# Autodesk Inventor assembly: 110033226_iam_02_造型房屋一
(part 2 of 2)
- 貼合:33 [Mate]: 110033226_ipt_06_磚塊樺木(1x1):1 ↔ 110033226_ipt_07_磚塊樺木(2x1):18
- 貼合:34 [Mate]: 110033226_ipt_07_磚塊樺木(2x1):23 ↔ 110033226_ipt_06_磚塊樺木(1x1):17
- 貼合:35 [Mate]: 110033226_ipt_07_磚塊樺木(2x1):23 ↔ 110033226_ipt_06_磚塊樺木(1x1):17
- 貼合:36 [Mate]: 110033226_ipt_07_磚塊樺木(2x1):23 ↔ 110033226_ipt_07_磚塊樺木(2x1):18
- 貼合:37 [Mate]: 110033226_ipt_06_磚塊樺木(1x1):22 ↔ 110033226_ipt_07_磚塊樺木(2x1):18
- 貼合:38 [Mate]: 110033226_ipt_06_磚塊樺木(1x1):22 ↔ 110033226_ipt_07_磚塊樺木(2x1):18
- 貼合:39 [Mate]: 110033226_ipt_07_磚塊樺木(2x1):25 ↔ 110033226_ipt_06_磚塊樺木(1x1):19
- 貼合:40 [Mate]: 110033226_ipt_07_磚塊樺木(2x1):25 ↔ 110033226_ipt_06_磚塊樺木(1x1):19
- 貼合:41 [Mate]: 110033226_ipt_06_磚塊樺木(1x1):24 ↔ 110033226_ipt_07_磚塊樺木(2x1):20
- 貼合:42 [Mate]: 110033226_ipt_06_磚塊樺木(1x1):24 ↔ 110033226_ipt_07_磚塊樺木(2x1):20
- 貼合:43 [Mate]: 110033226_ipt_06_磚塊樺木(1x1):2 ↔ 110033226_ipt_07_磚塊樺木(2x1):21
- 貼合:44 [Mate]: 110033226_ipt_07_磚塊樺木(2x1):2 ↔ 110033226_ipt_06_磚塊樺木(1x1):25
- 貼合:45 [Mate]: 110033226_ipt_06_磚塊樺木(1x1):2 ↔ 110033226_ipt_07_磚塊樺木(2x1):21
- 貼合:46 [Mate]: 110033226_ipt_07_磚塊樺木(2x1):2 ↔ 110033226_ipt_07_磚塊樺木(2x1):21
- 貼合:47 [Mate]: 110033226_ipt_07_磚塊樺木(2x1):2 ↔ 110033226_ipt_06_磚塊樺木(1x1):25
- 貼合:48 [Mate]: 110033226_ipt_06_磚塊樺木(1x1):10 ↔ 110033226_ipt_07_磚塊樺木(2x1):22
- 貼合:49 [Mate]: 110033226_ipt_07_磚塊樺木(2x1):10 ↔ 110033226_ipt_07_磚塊樺木(2x1):22
- 貼合:50 [Mate]: 110033226_ipt_06_磚塊樺木(1x1):10 ↔ 110033226_ipt_07_磚塊樺木(2x1):22
- 貼合:51 [Mate]: 110033226_ipt_06_磚塊樺木(1x1):25 ↔ 110033226_ipt_07_磚塊樺木(2x1):24
- 貼合:52 [Mate]: 110033226_ipt_06_磚塊樺木(1x1):25 ↔ 110033226_ipt_07_磚塊樺木(2x1):24
- 貼合:53 [Mate]: 110033226_ipt_07_磚塊樺木(2x1):21 ↔ 110033226_ipt_07_磚塊樺木(2x1):24
- 貼合:54 [Mate]: 110033226_ipt_07_磚塊樺木(2x1):10 ↔ 110033226_ipt_06_磚塊樺木(1x1):20
- 貼合:55 [Mate]: 110033226_ipt_07_磚塊樺木(2x1):10 ↔ 110033226_ipt_06_磚塊樺木(1x1):20
- 貼合:56 [Mate]: 110033226_ipt_07_磚塊樺木(2x1):21 ↔ 110033226_ipt_06_磚塊樺木(1x1):21
- 貼合:57 [Mate]: 110033226_ipt_07_磚塊樺木(2x1):21 ↔ 110033226_ipt_06_磚塊樺木(1x1):21
- 貼合:58 [Mate]: 110033226_ipt_06_磚塊樺木(1x1):22 ↔ 110033226_ipt_07_磚塊樺木(2x1):26
- 貼合:59 [Mate]: 110033226_ipt_06_磚塊樺木(1x1):22 ↔ 110033226_ipt_07_磚塊樺木(2x1):26
- 貼合:60 [Mate]: 110033226_ipt_07_磚塊樺木(2x1):23 ↔ 110033226_ipt_07_磚塊樺木(2x1):26
- 貼合:61 [Mate]: 110033226_ipt_07_磚塊樺木(2x1):23 ↔ 110033226_ipt_06_磚塊樺木(1x1):23
- 貼合:62 [Mate]: 110033226_ipt_07_磚塊樺木(2x1):23 ↔ 110033226_ipt_06_磚塊樺木(1x1):23
- 貼合:63 [Mate]: 110033226_ipt_06_磚塊樺木(1x1):20 ↔ 110033226_ipt_07_磚塊樺木(2x1):46
- 貼合:64 [Mate]: 110033226_ipt_06_磚塊樺木(1x1):20 ↔ 110033226_ipt_07_磚塊樺木(2x1):46
- 貼合:65 [Mate]: 110033226_ipt_07_磚塊樺木(2x1):22 ↔ 110033226_ipt_07_磚塊樺木(2x1):46
- 貼合:66 [Mate]: 110033226_ipt_07_磚塊樺木(2x1):22 ↔ 110033226_ipt_06_磚塊樺木(1x1):43
- 貼合:67 [Mate]: 110033226_ipt_07_磚塊樺木(2x1):22 ↔ 110033226_ipt_06_磚塊樺木(1x1):43
- 貼合:68 [Mate]: 110033226_ipt_06_磚塊樺木(1x1):24 ↔ 110033226_ipt_07_磚塊樺木(2x1):25
- 貼合:69 [Mate]: 110033226_ipt_06_磚塊樺木(1x1):22 ↔ 110033226_ipt_06_磚塊樺木(1x1):18
- 貼合:70 [Mate]: 110033226_ipt_06_磚塊樺木(1x1):17 ↔ 110033226_ipt_07_磚塊樺木(2x1):18
- 貼合:71 [Mate]: 110033226_ipt_06_磚塊樺木(1x1):23 ↔ 110033226_ipt_07_磚塊樺木(2x1):26
- 貼合:72 [Mate]: 110033226_ipt_06_磚塊樺木(1x1):43 ↔ 110033226_ipt_07_磚塊樺木(2x1):46
- 貼合:73 [Mate]: 110033226_ipt_07_磚塊樺木(2x1):46 ↔ 110033226_ipt_06_磚塊樺木(1x1):42
- 貼合:74 [Mate]: 110033226_ipt_07_磚塊樺木(2x1):46 ↔ 110033226_ipt_06_磚塊樺木(1x1):42
- 貼合:75 [Mate]: 110033226_ipt_07_磚塊樺木(2x1):46 ↔ 110033226_ipt_07_磚塊樺木(2x1):44
- 貼合:76 [Mate]: 110033226_ipt_07_磚塊樺木(2x1):46 ↔ 110033226_ipt_07_磚塊樺木(2x1):44
- 貼合:77 [Mate]: 110033226_ipt_06_磚塊樺木(1x1):43 ↔ 110033226_ipt_07_磚塊樺木(2x1):44
- 貼合:78 [Mate]: 110033226_ipt_07_磚塊樺木(2x1):44 ↔ 110033226_ipt_06_磚塊樺木(1x1):42
- 貼合:79 [Mate]: 110033226_ipt_06_磚塊樺木(1x1):42 ↔ 110033226_ipt_07_磚塊樺木(2x1):43
- 貼合:80 [Mate]: 110033226_ipt_07_磚塊樺木(2x1):44 ↔ 110033226_ipt_07_磚塊樺木(2x1):43
- 貼合:81 [Mate]: 110033226_ipt_06_磚塊樺木(1x1):42 ↔ 110033226_ipt_07_磚塊樺木(2x1):43
- 貼合:82 [Mate]: 110033226_ipt_07_磚塊樺木(2x1):44 ↔ 110033226_ipt_06_磚塊樺木(1x1):44
- 貼合:83 [Mate]: 110033226_ipt_07_磚塊樺木(2x1):44 ↔ 110033226_ipt_06_磚塊樺木(1x1):44
- 貼合:84 [Mate]: 110033226_ipt_07_磚塊樺木(2x1):43 ↔ 110033226_ipt_07_磚塊樺木(2x1):45
- 貼合:85 [Mate]: 110033226_ipt_07_磚塊樺木(2x1):43 ↔ 110033226_ipt_07_磚塊樺木(2x1):45
- 貼合:86 [Mate]: 110033226_ipt_06_磚塊樺木(1x1):44 ↔ 110033226_ipt_07_磚塊樺木(2x1):45
- 貼合:87 [Mate]: 110033226_ipt_06_磚塊樺木(1x1):62 ↔ 110033226_ipt_07_磚塊樺木(2x1):52
- 貼合:88 [Mate]: 110033226_ipt_07_磚塊樺木(2x1):63 ↔ 110033226_ipt_07_磚塊樺木(2x1):52
- 貼合:89 [Mate]: 110033226_ipt_06_磚塊樺木(1x1):62 ↔ 110033226_ipt_07_磚塊樺木(2x1):52
- 貼合:93 [Mate]: 110033226_ipt_08_平滑面(3x1):3 ↔ 110033226_ipt_07_磚塊樺木(2x1):19
- 貼合:94 [Mate]: 110033226_ipt_08_平滑面(3x1):3 ↔ 110033226_ipt_07_磚塊樺木(2x1):19
- 貼合:95 [Mate]: 110033226_ipt_08_平滑面(3x1):3 ↔ 110033226_ipt_06_磚塊樺木(1x1):18
- 貼合:96 [Mate]: 110033226_ipt_07_磚塊樺木(2x1):63 ↔ 110033226_ipt_06_磚塊樺木(1x1):45
- 貼合:97 [Mate]: 110033226_ipt_07_磚塊樺木(2x1):63 ↔ 110033226_ipt_06_磚塊樺木(1x1):45
- 貼合:98 [Mate]: 110033226_ipt_07_磚塊樺木(2x1):52 ↔ 110033226_ipt_06_磚塊樺木(1x1):45
- 貼合:99 [Mate]: 110033226_ipt_07_磚塊樺木(2x1):52 ↔ 110033226_ipt_07_磚塊樺木(2x1):51
- 貼合:100 [Mate]: 110033226_ipt_06_磚塊樺木(1x1):45 ↔ 110033226_ipt_07_磚塊樺木(2x1):51
- 貼合:101 [Mate]: 110033226_ipt_07_磚塊樺木(2x1):52 ↔ 110033226_ipt_07_磚塊樺木(2x1):51
- 貼合:102 [Mate]: 110033226_ipt_07_磚塊樺木(2x1):43 ↔ 110033226_ipt_06_磚塊樺木(1x1):51
- 貼合:103 [Mate]: 110033226_ipt_07_磚塊樺木(2x1):43 ↔ 110033226_ipt_06_磚塊樺木(1x1):51
- 貼合:104 [Mate]: 110033226_ipt_07_磚塊樺木(2x1):51 ↔ 110033226_ipt_06_磚塊樺木(1x1):51
- 貼合:105 [Mate]: 110033226_ipt_07_磚塊樺木(2x1):52 ↔ 110033226_ipt_06_磚塊樺木(1x1):47
- 貼合:106 [Mate]: 110033226_ipt_07_磚塊樺木(2x1):52 ↔ 110033226_ipt_06_磚塊樺木(1x1):47
- 貼合:107 [Mate]: 110033226_ipt_06_磚塊樺木(1x1):47 ↔ 110033226_ipt_07_磚塊樺木(2x1):51
- 貼合:111 [Mate]: 110033226_ipt_07_磚塊樺木(2x1):51 ↔ 110033226_ipt_07_磚塊樺木(2x1):47
- 貼合:112 [Mate]: 110033226_ipt_07_磚塊樺木(2x1):51 ↔ 110033226_ipt_07_磚塊樺木(2x1):47
- 貼合:113 [Mate]: 110033226_ipt_06_磚塊樺木(1x1):47 ↔ 110033226_ipt_07_磚塊樺木(2x1):47
- 貼合:114 [Mate]: 110033226_ipt_07_磚塊樺木(2x1):51 ↔ 110033226_ipt_06_磚塊樺木(1x1):46
- 貼合:115 [Mate]: 110033226_ipt_07_磚塊樺木(2x1):51 ↔ 110033226_ipt_06_磚塊樺木(1x1):46
- 貼合:116 [Mate]: 110033226_ipt_07_磚塊樺木(2x1):47 ↔ 110033226_ipt_06_磚塊樺木(1x1):46
- 貼合:117 [Mate]: 110033226_ipt_09_窗戶圓拱:1 ↔ 110033226_ipt_07_磚塊樺木(2x1):47
- 貼合:118 [Mate]: 110033226_ipt_09_窗戶圓拱:1 ↔ 110033226_ipt_06_磚塊樺木(1x1):65
- 貼合:119 [Mate]: 110033226_ipt_09_窗戶圓拱:1 ↔ 110033226_ipt_06_磚塊樺木(1x1):65
- 貼合:120 [Mate]: 110033226_ipt_06_磚塊樺木(1x1):51 ↔ 110033226_ipt_07_磚塊樺木(2x1):49
- 貼合:121 [Mate]: 110033226_ipt_06_磚塊樺木(1x1):51 ↔ 110033226_ipt_07_磚塊樺木(2x1):49
- 貼合:122 [Mate]: 110033226_ipt_07_磚塊樺木(2x1):49 ↔ 110033226_ipt_07_磚塊樺木(2x1):45
- 貼合:123 [Mate]: 110033226_ipt_06_磚塊樺木(1x1):48 ↔ 110033226_ipt_07_磚塊樺木(2x1):45
- 貼合:124 [Mate]: 110033226_ipt_06_磚塊樺木(1x1):48 ↔ 110033226_ipt_07_磚塊樺木(2x1):45
- 貼合:125 [Mate]: 110033226_ipt_07_磚塊樺木(2x1):49 ↔ 110033226_ipt_06_磚塊樺木(1x1):48
- 貼合:126 [Mate]: 110033226_ipt_06_磚塊樺木(1x1):48 ↔ 110033226_ipt_07_磚塊樺木(2x1):70
- 貼合:127 [Mate]: 110033226_ipt_07_磚塊樺木(2x1):49 ↔ 110033226_ipt_07_磚塊樺木(2x1):70
- 貼合:128 [Mate]: 110033226_ipt_06_磚塊樺木(1x1):48 ↔ 110033226_ipt_07_磚塊樺木(2x1):70
- 貼合:129 [Mate]: 110033226_ipt_07_磚塊樺木(2x1):49 ↔ 110033226_ipt_06_磚塊樺木(1x1):74
- 貼合:130 [Mate]: 110033226_ipt_06_磚塊樺木(1x1):74 ↔ 110033226_ipt_07_磚塊樺木(2x1):70
- 貼合:131 [Mate]: 110033226_ipt_07_磚塊樺木(2x1):49 ↔ 110033226_ipt_06_磚塊樺木(1x1):74
- 貼合:132 [Mate]: 110033226_ipt_06_磚塊樺木(1x1):46 ↔ 110033226_ipt_07_磚塊樺木(2x1):75
- 貼合:133 [Mate]: 110033226_ipt_06_磚塊樺木(1x1):46 ↔ 110033226_ipt_07_磚塊樺木(2x1):75
- 貼合:134 [Mate]: 110033226_ipt_07_磚塊樺木(2x1):47 ↔ 110033226_ipt_07_磚塊樺木(2x1):75
- 貼合:135 [Mate]: 110033226_ipt_06_磚塊樺木(1x1):74 ↔ 110033226_ipt_07_磚塊樺木(2x1):79
- 貼合:136 [Mate]: 110033226_ipt_06_磚塊樺木(1x1):74 ↔ 110033226_ipt_07_磚塊樺木(2x1):79
- 貼合:137 [Mate]: 110033226_ipt_07_磚塊樺木(2x1):79 ↔ 110033226_ipt_07_磚塊樺木(2x1):70
- 貼合:138 [Mate]: 110033226_ipt_06_磚塊樺木(1x1):76 ↔ 110033226_ipt_07_磚塊樺木(2x1):70
- 貼合:139 [Mate]: 110033226_ipt_06_磚塊樺木(1x1):76 ↔ 110033226_ipt_07_磚塊樺木(2x1):70
- 貼合:140 [Mate]: 110033226_ipt_07_磚塊樺木(2x1):79 ↔ 110033226_ipt_06_磚塊樺木(1x1):76
- 貼合:141 [Mate]: 110033226_ipt_07_磚塊樺木(2x1):75 ↔ 110033226_ipt_07_磚塊樺木(2x1):78
- 貼合:142 [Mate]: 110033226_ipt_07_磚塊樺木(2x1):75 ↔ 110033226_ipt_07_磚塊樺木(2x1):78
- 貼合:143 [Mate]: 110033226_ipt_07_磚塊樺木(2x1):75 ↔ 110033226_ipt_07_磚塊樺木(2x1):78
- 貼合:144 [Mate]: 110033226_ipt_07_磚塊樺木(2x1):78 ↔ 110033226_ipt_07_磚塊樺木(2x1):73
- 貼合:145 [Mate]: 110033226_ipt_07_磚塊樺木(2x1):78 ↔ 110033226_ipt_07_磚塊樺木(2x1):73
- 貼合:146 [Mate]: 110033226_ipt_07_磚塊樺木(2x1):78 ↔ 110033226_ipt_07_磚塊樺木(2x1):73
- 貼合:147 [Mate]: 110033226_ipt_07_磚塊樺木(2x1):73 ↔ 110033226_ipt_07_磚塊樺木(2x1):72
- 貼合:148 [Mate]: 110033226_ipt_07_磚塊樺木(2x1):73 ↔ 110033226_ipt_07_磚塊樺木(2x1):72
- 貼合:149 [Mate]: 110033226_ipt_07_磚塊樺木(2x1):73 ↔ 110033226_ipt_07_磚塊樺木(2x1):72
- 貼合:150 [Mate]: 110033226_ipt_07_磚塊樺木(2x1):72 ↔ 110033226_ipt_06_磚塊樺木(1x1):71
- 貼合:151 [Mate]: 110033226_ipt_07_磚塊樺木(2x1):72 ↔ 110033226_ipt_06_磚塊樺木(1x1):71
- 貼合:152 [Mate]: 110033226_ipt_09_窗戶圓拱:1 ↔ 110033226_ipt_07_磚塊樺木(2x1):74
- 貼合:153 [Mate]: 110033226_ipt_07_磚塊樺木(2x1):72 ↔ 110033226_ipt_07_磚塊樺木(2x1):74
- 貼合:154 [Mate]: 110033226_ipt_07_磚塊樺木(2x1):74 ↔ 110033226_ipt_06_磚塊樺木(1x1):71
- 貼合:155 [Mate]: 110033226_ipt_07_磚塊樺木(2x1):74 ↔ 110033226_ipt_08_平滑面(3x1):2
- 貼合:156 [Mate]: 110033226_ipt_06_磚塊樺木(1x1):71 ↔ 110033226_ipt_08_平滑面(3x1):2
- 貼合:157 [Mate]: 110033226_ipt_07_磚塊樺木(2x1):74 ↔ 110033226_ipt_08_平滑面(3x1):2
- 對稱:1 [Symmetry]: 110033226_ipt_06_磚塊樺木(1x1):76 ↔ 110033226_ipt_07_磚塊樺木(2x1):67
- 貼合:158 [Mate]: 110033226_ipt_07_磚塊樺木(2x1):79 ↔ 110033226_ipt_07_磚塊樺木(2x1):67
- 貼合:159 [Mate]: 110033226_ipt_06_磚塊樺木(1x1):76 ↔ 110033226_ipt_07_磚塊樺木(2x1):67
- 貼合:160 [Mate]: 110033226_ipt_07_磚塊樺木(2x1):79 ↔ 110033226_ipt_06_磚塊樺木(1x1):69
- 貼合:161 [Mate]: 110033226_ipt_07_磚塊樺木(2x1):79 ↔ 110033226_ipt_06_磚塊樺木(1x1):69
- 角度:1 [Angle] (0 deg): 110033226_ipt_07_磚塊樺木(2x1):67 ↔ 110033226_ipt_06_磚塊樺木(1x1):69
- 貼合:162 [Mate]: 110033226_ipt_07_磚塊樺木(2x1):71 ↔ 110033226_ipt_06_磚塊樺木(1x1):69
- 貼合:163 [Mate]: 110033226_ipt_07_磚塊樺木(2x1):67 ↔ 110033226_ipt_07_磚塊樺木(2x1):71
- 貼合:164 [Mate]: 110033226_ipt_07_磚塊樺木(2x1):71 ↔ 110033226_ipt_06_磚塊樺木(1x1):69
- 貼合:165 [Mate]: 110033226_ipt_07_磚塊樺木(2x1):67 ↔ 110033226_ipt_06_磚塊樺木(1x1):70
- 貼合:166 [Mate]: 110033226_ipt_07_磚塊樺木(2x1):67 ↔ 110033226_ipt_06_磚塊樺木(1x1):70
- 貼合:167 [Mate]: 110033226_ipt_06_磚塊樺木(1x1):70 ↔ 110033226_ipt_07_磚塊樺木(2x1):71
- 貼合:168 [Mate]: 110033226_ipt_06_磚塊樺木(1x1):70 ↔ 110033226_ipt_08_平滑面(3x1):5
- 貼合:169 [Mate]: 110033226_ipt_07_磚塊樺木(2x1):71 ↔ 110033226_ipt_08_平滑面(3x1):5
- 貼合:170 [Mate]: 110033226_ipt_06_磚塊樺木(1x1):70 ↔ 110033226_ipt_08_平滑面(3x1):5
- 貼合:171 [Mate]: 110033226_ipt_10_木板條:2 ↔ 110033226_ipt_07_磚塊樺木(2x1):71
- 貼合:172 [Mate]: 110033226_ipt_10_木板條:2 ↔ 110033226_ipt_08_平滑面(3x1):5
- 貼合:173 [Mate]: 110033226_ipt_05_房子底座:1 ↔ 110033226_ipt_10_木板條:2
- 貼合:174 [Mate]: 110033226_ipt_10_木板條:2 ↔ 110033226_ipt_11_樓梯支架:1
- 貼合:175 [Mate]: 110033226_ipt_10_木板條:2 ↔ 110033226_ipt_11_樓梯支架:1
- 貼合:176 [Mate]: 110033226_ipt_10_木板條:2 ↔ 110033226_ipt_11_樓梯支架:1
- 貼合:177 [Mate]: 110033226_ipt_10_木板條:3 ↔ 110033226_ipt_11_樓梯支架:1
- 貼合:178 [Mate]: 110033226_ipt_10_木板條:3 ↔ 110033226_ipt_11_樓梯支架:7
- 貼合:179 [Mate]: 110033226_ipt_10_木板條:3 ↔ 110033226_ipt_11_樓梯支架:1
- 貼合:180 [Mate]: 110033226_ipt_10_木板條:7 ↔ 110033226_ipt_11_樓梯支架:8
- 貼合:181 [Mate]: 110033226_ipt_10_木板條:5 ↔ 110033226_ipt_11_樓梯支架:6
- 貼合:182 [Mate]: 110033226_ipt_10_木板條:4 ↔ 110033226_ipt_11_樓梯支架:5
- 貼合:183 [Mate]: 110033226_ipt_10_木板條:6 ↔ 110033226_ipt_11_樓梯支架:4
- 貼合:184 [Mate]: 110033226_ipt_10_木板條:5 ↔ 110033226_ipt_11_樓梯支架:6
- 貼合:185 [Mate]: 110033226_ipt_10_木板條:5 ↔ 110033226_ipt_11_樓梯支架:11
- 貼合:186 [Mate]: 110033226_ipt_10_木板條:4 ↔ 110033226_ipt_11_樓梯支架:10
- 貼合:187 [Mate]: 110033226_ipt_10_木板條:4 ↔ 110033226_ipt_11_樓梯支架:5
- 貼合:188 [Mate]: 110033226_ipt_10_木板條:6 ↔ 110033226_ipt_11_樓梯支架:4
- 貼合:189 [Mate]: 110033226_ipt_10_木板條:6 ↔ 110033226_ipt_11_樓梯支架:9
- 貼合:190 [Mate]: 110033226_ipt_10_木板條:7 ↔ 110033226_ipt_11_樓梯支架:3
- 貼合:191 [Mate]: 110033226_ipt_10_木板條:7 ↔ 110033226_ipt_11_樓梯支架:8
- 貼合:192 [Mate]: 110033226_ipt_06_磚塊樺木(1x1):16 ↔ 110033226_ipt_07_磚塊樺木(2x1):16
- 貼合:193 [Mate]: 110033226_ipt_06_磚塊樺木(1x1):171 ↔ 110033226_ipt_08_平滑面(3x1):1
- 貼合:194 [Mate]: 110033226_ipt_07_磚塊樺木(2x1):187 ↔ 110033226_ipt_08_平滑面(3x1):1
- 貼合:195 [Mate]: 110033226_ipt_06_磚塊樺木(1x1):171 ↔ 110033226_ipt_08_平滑面(3x1):1
- 貼合:196 [Mate]: 110033226_ipt_07_磚塊樺木(2x1):188 ↔ 110033226_ipt_08_平滑面(3x1):4
- 貼合:197 [Mate]: 110033226_ipt_07_磚塊樺木(2x1):188 ↔ 110033226_ipt_08_平滑面(3x1):4
- 貼合:198 [Mate]: 110033226_ipt_08_平滑面(3x1):4 ↔ 110033226_ipt_08_平滑面(3x1):17
- 貼合:199 [Mate]: 110033226_ipt_06_磚塊樺木(1x1):66 ↔ 110033226_ipt_08_平滑面(3x1):9
- 貼合:200 [Mate]: 110033226_ipt_06_磚塊樺木(1x1):66 ↔ 110033226_ipt_08_平滑面(3x1):9
- 貼合:201 [Mate]: 110033226_ipt_06_磚塊樺木(1x1):66 ↔ 110033226_ipt_08_平滑面(3x1):9
- 貼合:202 [Mate]: 110033226_ipt_07_磚塊樺木(2x1):69 ↔ 110033226_ipt_08_平滑面(3x1):9
- 貼合:203 [Mate]: 110033226_ipt_06_磚塊樺木(1x1):66 ↔ 110033226_ipt_07_磚塊樺木(2x1):69
- 貼合:204 [Mate]: 110033226_ipt_07_磚塊樺木(2x1):69 ↔ 110033226_ipt_08_平滑面(3x1):11
- 貼合:205 [Mate]: 110033226_ipt_07_磚塊樺木(2x1):76 ↔ 110033226_ipt_06_磚塊樺木(1x1):66
- 貼合:206 [Mate]: 110033226_ipt_07_磚塊樺木(2x1):76 ↔ 110033226_ipt_06_磚塊樺木(1x1):66
- 貼合:207 [Mate]: 110033226_ipt_07_磚塊樺木(2x1):76 ↔ 110033226_ipt_07_磚塊樺木(2x1):69
- 貼合:208 [Mate]: 110033226_ipt_06_磚塊樺木(1x1):73 ↔ 110033226_ipt_07_磚塊樺木(2x1):69
- 貼合:209 [Mate]: 110033226_ipt_06_磚塊樺木(1x1):73 ↔ 110033226_ipt_07_磚塊樺木(2x1):69
- 貼合:210 [Mate]: 110033226_ipt_07_磚塊樺木(2x1):76 ↔ 110033226_ipt_06_磚塊樺木(1x1):73
- 貼合:211 [Mate]: 110033226_ipt_08_平滑面(3x1):2 ↔ 110033226_ipt_07_磚塊樺木(2x1):68
- 貼合:212 [Mate]: 110033226_ipt_08_平滑面(3x1):2 ↔ 110033226_ipt_07_磚塊樺木(2x1):68
- 貼合:213 [Mate]: 110033226_ipt_08_平滑面(3x1):2 ↔ 110033226_ipt_07_磚塊樺木(2x1):68
- 貼合:214 [Mate]: 110033226_ipt_08_平滑面(3x1):2 ↔ 110033226_ipt_06_磚塊樺木(1x1):75
- 貼合:215 [Mate]: 110033226_ipt_07_磚塊樺木(2x1):68 ↔ 110033226_ipt_06_磚塊樺木(1x1):75
- 貼合:216 [Mate]: 110033226_ipt_08_平滑面(3x1):6 ↔ 110033226_ipt_06_磚塊樺木(1x1):75
- 貼合:217 [Mate]: 110033226_ipt_06_磚塊樺木(1x1):68 ↔ 110033226_ipt_08_平滑面(3x1):18
- 貼合:218 [Mate]: 110033226_ipt_06_磚塊樺木(1x1):68 ↔ 110033226_ipt_08_平滑面(3x1):18
- 貼合:219 [Mate]: 110033226_ipt_06_磚塊樺木(1x1):68 ↔ 110033226_ipt_08_平滑面(3x1):18
- 貼合:220 [Mate]: 110033226_ipt_07_磚塊樺木(2x1):209 ↔ 110033226_ipt_08_平滑面(3x1):18
- 貼合:221 [Mate]: 110033226_ipt_07_磚塊樺木(2x1):209 ↔ 110033226_ipt_08_平滑面(3x1):18
- 貼合:222 [Mate]: 110033226_ipt_06_磚塊樺木(1x1):68 ↔ 110033226_ipt_07_磚塊樺木(2x1):209
- 貼合:223 [Mate]: 110033226_ipt_06_磚塊樺木(1x1):68 ↔ 110033226_ipt_07_磚塊樺木(2x1):210
- 貼合:224 [Mate]: 110033226_ipt_06_磚塊樺木(1x1):68 ↔ 110033226_ipt_07_磚塊樺木(2x1):210
- 貼合:225 [Mate]: 110033226_ipt_07_磚塊樺木(2x1):210 ↔ 110033226_ipt_07_磚塊樺木(2x1):209
- 對稱:2 [Symmetry]: 110033226_ipt_06_磚塊樺木(1x1):192 ↔ 110033226_ipt_07_磚塊樺木(2x1):209
- 貼合:226 [Mate]: 110033226_ipt_07_磚塊樺木(2x1):210 ↔ 110033226_ipt_06_磚塊樺木(1x1):192
- 貼合:227 [Mate]: 110033226_ipt_06_磚塊樺木(1x1):192 ↔ 110033226_ipt_07_磚塊樺木(2x1):209
- 貼合:228 [Mate]: 110033226_ipt_07_磚塊樺木(2x1):68 ↔ 110033226_ipt_07_磚塊樺木(2x1):239
- 貼合:229 [Mate]: 110033226_ipt_06_磚塊樺木(1x1):75 ↔ 110033226_ipt_07_磚塊樺木(2x1):239
- 貼合:230 [Mate]: 110033226_ipt_07_磚塊樺木(2x1):68 ↔ 110033226_ipt_07_磚塊樺木(2x1):239
- 貼合:231 [Mate]: 110033226_ipt_07_磚塊樺木(2x1):68 ↔ 110033226_ipt_06_磚塊樺木(1x1):221
- 貼合:232 [Mate]: 110033226_ipt_07_磚塊樺木(2x1):68 ↔ 110033226_ipt_06_磚塊樺木(1x1):221
- 貼合:233 [Mate]: 110033226_ipt_07_磚塊樺木(2x1):239 ↔ 110033226_ipt_06_磚塊樺木(1x1):221
- 貼合:234 [Mate]: 110033226_ipt_06_磚塊樺木(1x1):221 ↔ 110033226_ipt_07_磚塊樺木(2x1):240
- 貼合:235 [Mate]: 110033226_ipt_06_磚塊樺木(1x1):221 ↔ 110033226_ipt_07_磚塊樺木(2x1):240
- 貼合:236 [Mate]: 110033226_ipt_07_磚塊樺木(2x1):239 ↔ 110033226_ipt_07_磚塊樺木(2x1):240
- 貼合:237 [Mate]: 110033226_ipt_06_磚塊樺木(1x1):222 ↔ 110033226_ipt_07_磚塊樺木(2x1):239
- 貼合:238 [Mate]: 110033226_ipt_06_磚塊樺木(1x1):222 ↔ 110033226_ipt_07_磚塊樺木(2x1):239
- 貼合:239 [Mate]: 110033226_ipt_06_磚塊樺木(1x1):222 ↔ 110033226_ipt_07_磚塊樺木(2x1):240
- 貼合:240 [Mate]: 110033226_ipt_07_磚塊樺木(2x1):257 ↔ 110033226_ipt_07_磚塊樺木(2x1):244
- 貼合:241 [Mate]: 110033226_ipt_07_磚塊樺木(2x1):257 ↔ 110033226_ipt_07_磚塊樺木(2x1):244
- 貼合:242 [Mate]: 110033226_ipt_07_磚塊樺木(2x1):257 ↔ 110033226_ipt_07_磚塊樺木(2x1):244
- 貼合:243 [Mate]: 110033226_ipt_07_磚塊樺木(2x1):257 ↔ 110033226_ipt_06_磚塊樺木(1x1):240
- 貼合:244 [Mate]: 110033226_ipt_07_磚塊樺木(2x1):257 ↔ 110033226_ipt_06_磚塊樺木(1x1):240
- 貼合:245 [Mate]: 110033226_ipt_07_磚塊樺木(2x1):257 ↔ 110033226_ipt_06_磚塊樺木(1x1):240
- 貼合:246 [Mate]: 110033226_ipt_06_磚塊樺木(1x1):239 ↔ 110033226_ipt_06_磚塊樺木(1x1):240
- 貼合:247 [Mate]: 110033226_ipt_06_磚塊樺木(1x1):239 ↔ 110033226_ipt_06_磚塊樺木(1x1):240
- 貼合:248 [Mate]: 110033226_ipt_06_磚塊樺木(1x1):239 ↔ 110033226_ipt_06_磚塊樺木(1x1):240
- 貼合:249 [Mate]: 110033226_ipt_06_磚塊樺木(1x1):237 ↔ 110033226_ipt_07_磚塊樺木(2x1):258
- 貼合:250 [Mate]: 110033226_ipt_06_磚塊樺木(1x1):237 ↔ 110033226_ipt_07_磚塊樺木(2x1):258
- 貼合:251 [Mate]: 110033226_ipt_07_磚塊樺木(2x1):256 ↔ 110033226_ipt_07_磚塊樺木(2x1):258
- 貼合:252 [Mate]: 110033226_ipt_07_磚塊樺木(2x1):256 ↔ 110033226_ipt_06_磚塊樺木(1x1):241
- 貼合:253 [Mate]: 110033226_ipt_07_磚塊樺木(2x1):256 ↔ 110033226_ipt_06_磚塊樺木(1x1):241
- 貼合:254 [Mate]: 110033226_ipt_07_磚塊樺木(2x1):258 ↔ 110033226_ipt_06_磚塊樺木(1x1):241
- 貼合:255 [Mate]: 110033226_ipt_06_磚塊樺木(1x1):242 ↔ 110033226_ipt_07_磚塊樺木(2x1):258
- 貼合:256 [Mate]: 110033226_ipt_06_磚塊樺木(1x1):242 ↔ 110033226_ipt_07_磚塊樺木(2x1):258
- 貼合:257 [Mate]: 110033226_ipt_06_磚塊樺木(1x1):242 ↔ 110033226_ipt_07_磚塊樺木(2x1):258
- 貼合:258 [Mate]: 110033226_ipt_07_磚塊樺木(2x1):259 ↔ 110033226_ipt_07_磚塊樺木(2x1):258
- 貼合:259 [Mate]: 110033226_ipt_07_磚塊樺木(2x1):259 ↔ 110033226_ipt_06_磚塊樺木(1x1):241
- 貼合:260 [Mate]: 110033226_ipt_07_磚塊樺木(2x1):259 ↔ 110033226_ipt_06_磚塊樺木(1x1):241
- 貼合:261 [Mate]: 110033226_ipt_06_磚塊樺木(1x1):240 ↔ 110033226_ipt_07_磚塊樺木(2x1):260
- 貼合:262 [Mate]: 110033226_ipt_07_磚塊樺木(2x1):257 ↔ 110033226_ipt_07_磚塊樺木(2x1):260
- 貼合:263 [Mate]: 110033226_ipt_06_磚塊樺木(1x1):240 ↔ 110033226_ipt_07_磚塊樺木(2x1):260
- 貼合:264 [Mate]: 110033226_ipt_06_磚塊樺木(1x1):239 ↔ 110033226_ipt_06_磚塊樺木(1x1):249
- 貼合:265 [Mate]: 110033226_ipt_06_磚塊樺木(1x1):249 ↔ 110033226_ipt_07_磚塊樺木(2x1):203
- 貼合:266 [Mate]: 110033226_ipt_07_磚塊樺木(2x1):260 ↔ 110033226_ipt_06_磚塊樺木(1x1):249
- 貼合:267 [Mate]: 110033226_ipt_07_磚塊樺木(2x1):265 ↔ 110033226_ipt_08_平滑面(3x1):12
- 貼合:268 [Mate]: 110033226_ipt_08_平滑面(3x1):1 ↔ 110033226_ipt_07_磚塊樺木(2x1):265
- 貼合:269 [Mate]: 110033226_ipt_07_磚塊樺木(2x1):190 ↔ 110033226_ipt_07_磚塊樺木(2x1):265
- 貼合:270 [Mate]: 110033226_ipt_08_平滑面(3x1):1 ↔ 110033226_ipt_06_磚塊樺木(1x1):248
- 貼合:271 [Mate]: 110033226_ipt_08_平滑面(3x1):1 ↔ 110033226_ipt_06_磚塊樺木(1x1):248
- 貼合:272 [Mate]: 110033226_ipt_07_磚塊樺木(2x1):265 ↔ 110033226_ipt_06_磚塊樺木(1x1):248
- 對稱:3 [Symmetry]: 110033226_ipt_07_磚塊樺木(2x1):266 ↔ 110033226_ipt_06_磚塊樺木(1x1):248
- 貼合:273 [Mate]: 110033226_ipt_07_磚塊樺木(2x1):265 ↔ 110033226_ipt_07_磚塊樺木(2x1):266
- 貼合:274 [Mate]: 110033226_ipt_07_磚塊樺木(2x1):266 ↔ 110033226_ipt_06_磚塊樺木(1x1):248
- 貼合:275 [Mate]: 110033226_ipt_07_磚塊樺木(2x1):265 ↔ 110033226_ipt_06_磚塊樺木(1x1):247
- 貼合:276 [Mate]: 110033226_ipt_07_磚塊樺木(2x1):265 ↔ 110033226_ipt_06_磚塊樺木(1x1):247
- 貼合:277 [Mate]: 110033226_ipt_07_磚塊樺木(2x1):266 ↔ 110033226_ipt_06_磚塊樺木(1x1):247
- 貼合:278 [Mate]: 110033226_ipt_06_磚塊樺木(1x1):268 ↔ 110033226_ipt_08_平滑面(3x1):17
- 貼合:279 [Mate]: 110033226_ipt_06_磚塊樺木(1x1):258 ↔ 110033226_ipt_06_磚塊樺木(1x1):268
- 貼合:280 [Mate]: 110033226_ipt_06_磚塊樺木(1x1):251 ↔ 110033226_ipt_08_平滑面(3x1):33
- 貼合:281 [Mate]: 110033226_ipt_07_磚塊樺木(2x1):269 ↔ 110033226_ipt_08_平滑面(3x1):33
- 貼合:282 [Mate]: 110033226_ipt_07_磚塊樺木(2x1):269 ↔ 110033226_ipt_08_平滑面(3x1):33
- 貼合:283 [Mate]: 110033226_ipt_08_平滑面(3x1):35 ↔ 110033226_ipt_07_磚塊樺木(2x1):221
- 貼合:284 [Mate]: 110033226_ipt_08_平滑面(3x1):35 ↔ 110033226_ipt_06_磚塊樺木(1x1):204
- 貼合:285 [Mate]: 110033226_ipt_08_平滑面(3x1):35 ↔ 110033226_ipt_07_磚塊樺木(2x1):221
- 貼合:286 [Mate]: 110033226_ipt_08_平滑面(3x1):34 ↔ 110033226_ipt_07_磚塊樺木(2x1):16
- 貼合:287 [Mate]: 110033226_ipt_08_平滑面(3x1):34 ↔ 110033226_ipt_07_磚塊樺木(2x1):16
- 貼合:288 [Mate]: 110033226_ipt_08_平滑面(3x1):34 ↔ 110033226_ipt_06_磚塊樺木(1x1):16
- 貼合:289 [Mate]: 110033226_ipt_12_平滑面(2x1):1 ↔ 110033226_ipt_07_磚塊樺木(2x1):17
- 貼合:290 [Mate]: 110033226_ipt_12_平滑面(2x1):1 ↔ 110033226_ipt_07_磚塊樺木(2x1):17
- 貼合:291 [Mate]: 110033226_ipt_08_平滑面(3x1):34 ↔ 110033226_ipt_12_平滑面(2x1):1
- 貼合:292 [Mate]: 110033226_ipt_05_房子底座:1 ↔ 110033226_ipt_13_草地二:1
- 貼合:293 [Mate]: 110033226_ipt_05_房子底座:1 ↔ 110033226_ipt_13_草地二:1
- 貼合:294 [Mate]: 110033226_ipt_05_房子底座:1 ↔ 110033226_ipt_13_草地二:1
- 貼合:295 [Mate]: 110033226_ipt_05_房子底座:1 ↔ 110033226_ipt_13_草地二:2
- 貼合:296 [Mate]: 110033226_ipt_05_房子底座:1 ↔ 110033226_ipt_13_草地二:2
- 貼合:297 [Mate]: 110033226_ipt_05_房子底座:1 ↔ 110033226_ipt_13_草地二:2
- 貼合:298 [Mate]: 110033226_ipt_05_房子底座:1 ↔ 110033226_ipt_02_草地一:1
- 貼合:299 [Mate]: 110033226_ipt_05_房子底座:1 ↔ 110033226_ipt_02_草地一:1
- 貼合:300 [Mate]: 110033226_ipt_05_房子底座:1 ↔ 110033226_ipt_02_草地一:1
- 貼合:301 [Mate]: 110033226_ipt_05_房子底座:1 ↔ 110033226_ipt_13_草地二:3
- 貼合:302 [Mate]: 110033226_ipt_05_房子底座:1 ↔ 110033226_ipt_13_草地二:3
- 貼合:303 [Mate]: 110033226_ipt_05_房子底座:1 ↔ 110033226_ipt_13_草地二:3
- 貼合:307 [Mate]: 110033226_ipt_14_草地三:2 ↔ 110033226_ipt_13_草地二:11
- 貼合:308 [Mate]: 110033226_ipt_14_草地三:2 ↔ 110033226_ipt_13_草地二:11
- 貼合:309 [Mate]: 110033226_ipt_14_草地三:2 ↔ 110033226_ipt_13_草地二:11
- 貼合:310 [Mate]: 110033226_ipt_05_房子底座:1 ↔ 110033226_ipt_13_草地二:14
- 貼合:311 [Mate]: 110033226_ipt_05_房子底座:1 ↔ 110033226_ipt_13_草地二:14
- 貼合:312 [Mate]: 110033226_ipt_05_房子底座:1 ↔ 110033226_ipt_13_草地二:14
- 貼合:313 [Mate]: 110033226_ipt_14_草地三:3 ↔ 110033226_ipt_13_草地二:14
- 貼合:314 [Mate]: 110033226_ipt_14_草地三:3 ↔ 110033226_ipt_13_草地二:14
- 貼合:315 [Mate]: 110033226_ipt_14_草地三:2 ↔ 110033226_ipt_14_草地三:3
- 貼合:316 [Mate]: 110033226_ipt_13_草地二:10 ↔ 110033226_ipt_13_草地二:19
- 貼合:317 [Mate]: 110033226_ipt_13_草地二:11 ↔ 110033226_ipt_13_草地二:19
- 貼合:318 [Mate]: 110033226_ipt_13_草地二:10 ↔ 110033226_ipt_13_草地二:19
- 貼合:319 [Mate]: 110033226_ipt_14_草地三:4 ↔ 110033226_ipt_13_草地二:19
- 貼合:320 [Mate]: 110033226_ipt_14_草地三:2 ↔ 110033226_ipt_14_草地三:4
- 貼合:321 [Mate]: 110033226_ipt_14_草地三:4 ↔ 110033226_ipt_13_草地二:19
- 貼合:322 [Mate]: 110033226_ipt_14_草地三:8 ↔ 110033226_ipt_13_草地二:7
- 貼合:323 [Mate]: 110033226_ipt_14_草地三:8 ↔ 110033226_ipt_13_草地二:7
- 貼合:324 [Mate]: 110033226_ipt_14_草地三:8 ↔ 110033226_ipt_02_草地一:1
- 貼合:325 [Mate]: 110033226_ipt_14_草地三:6 ↔ 110033226_ipt_13_草地二:1
- 貼合:326 [Mate]: 110033226_ipt_14_草地三:6 ↔ 110033226_ipt_13_草地二:4
- 貼合:327 [Mate]: 110033226_ipt_14_草地三:6 ↔ 110033226_ipt_13_草地二:27
- 貼合:328 [Mate]: 110033226_ipt_14_草地三:9 ↔ 110033226_ipt_13_草地二:4
- 貼合:329 [Mate]: 110033226_ipt_14_草地三:6 ↔ 110033226_ipt_14_草地三:9
- 貼合:330 [Mate]: 110033226_ipt_14_草地三:9 ↔ 110033226_ipt_13_草地二:4
- 貼合:331 [Mate]: 110033226_ipt_13_草地二:20 ↔ 110033226_ipt_13_草地二:4
- 貼合:332 [Mate]: 110033226_ipt_13_草地二:20 ↔ 110033226_ipt_13_草地二:4
- 貼合:333 [Mate]: 110033226_ipt_13_草地二:20 ↔ 110033226_ipt_13_草地二:5
- 貼合:334 [Mate]: 110033226_ipt_13_草地二:20 ↔ 110033226_ipt_14_草地三:7
- 貼合:335 [Mate]: 110033226_ipt_13_草地二:20 ↔ 110033226_ipt_14_草地三:7
- 對稱:4 [Symmetry]: 110033226_ipt_13_草地二:20 ↔ 110033226_ipt_14_草地三:7
- 貼合:336 [Mate]: 110033226_ipt_14_草地三:5 ↔ 110033226_ipt_13_草地二:19
- 貼合:337 [Mate]: 110033226_ipt_14_草地三:5 ↔ 110033226_ipt_13_草地二:19
- 貼合:338 [Mate]: 110033226_ipt_14_草地三:4 ↔ 110033226_ipt_14_草地三:5
- 貼合:339 [Mate]: 110033226_ipt_13_草地二:22 ↔ 110033226_ipt_13_草地二:24
- 貼合:340 [Mate]: 110033226_ipt_13_草地二:22 ↔ 110033226_ipt_13_草地二:24
- 貼合:341 [Mate]: 110033226_ipt_13_草地二:22 ↔ 110033226_ipt_13_草地二:24
- 貼合:342 [Mate]: 110033226_ipt_14_草地三:12 ↔ 110033226_ipt_13_草地二:25
- 貼合:343 [Mate]: 110033226_ipt_13_草地二:22 ↔ 110033226_ipt_14_草地三:12
- 貼合:344 [Mate]: 110033226_ipt_14_草地三:10 ↔ 110033226_ipt_13_草地二:25
- 貼合:345 [Mate]: 110033226_ipt_14_草地三:10 ↔ 110033226_ipt_13_草地二:25
- 貼合:346 [Mate]: 110033226_ipt_14_草地三:10 ↔ 110033226_ipt_14_草地三:12
- 貼合:347 [Mate]: 110033226_ipt_14_草地三:13 ↔ 110033226_ipt_13_草地二:26
- 貼合:348 [Mate]: 110033226_ipt_14_草地三:13 ↔ 110033226_ipt_13_草地二:26
- 貼合:349 [Mate]: 110033226_ipt_14_草地三:10 ↔ 110033226_ipt_14_草地三:13
- 貼合:350 [Mate]: 110033226_ipt_14_草地三:11 ↔ 110033226_ipt_13_草地二:26
- 貼合:351 [Mate]: 110033226_ipt_14_草地三:11 ↔ 110033226_ipt_13_草地二:26
- 貼合:352 [Mate]: 110033226_ipt_14_草地三:11 ↔ 110033226_ipt_14_草地三:13
- 貼合:353 [Mate]: 110033226_ipt_13_草地二:23 ↔ 110033226_ipt_13_草地二:27
- 貼合:354 [Mate]: 110033226_ipt_13_草地二:23 ↔ 110033226_ipt_13_草地二:27
- 貼合:355 [Mate]: 110033226_ipt_13_草地二:23 ↔ 110033226_ipt_13_草地二:27
- 貼合:356 [Mate]: 110033226_ipt_13_草地二:21 ↔ 110033226_ipt_13_草地二:23
- 貼合:357 [Mate]: 110033226_ipt_13_草地二:21 ↔ 110033226_ipt_13_草地二:23
- 貼合:358 [Mate]: 110033226_ipt_13_草地二:21 ↔ 110033226_ipt_13_草地二:23
- 貼合:361 [Mate]: 110033226_ipt_13_草地二:21 ↔ 110033226_ipt_14_草地三:14
- 貼合:363 [Mate]: 110033226_ipt_13_草地二:21 ↔ 110033226_ipt_14_草地三:14
- 貼合:364 [Mate]: 110033226_ipt_13_草地二:21 ↔ 110033226_ipt_14_草地三:14
- 貼合:365 [Mate]: 110033226_ipt_14_草地三:16 ↔ 110033226_ipt_13_草地二:7
- 貼合:366 [Mate]: 110033226_ipt_14_草地三:16 ↔ 110033226_ipt_13_草地二:7
- 貼合:367 [Mate]: 110033226_ipt_14_草地三:8 ↔ 110033226_ipt_14_草地三:16
- 貼合:368 [Mate]: 110033226_ipt_14_草地三:7 ↔ 110033226_ipt_14_草地三:17
- 貼合:369 [Mate]: 110033226_ipt_13_草地二:20 ↔ 110033226_ipt_14_草地三:17
- 貼合:370 [Mate]: 110033226_ipt_13_草地二:20 ↔ 110033226_ipt_14_草地三:17
- 貼合:371 [Mate]: 110033226_ipt_13_草地二:13 ↔ 110033226_ipt_02_草地一:2
- 貼合:372 [Mate]: 110033226_ipt_13_草地二:13 ↔ 110033226_ipt_02_草地一:2
- 貼合:373 [Mate]: 110033226_ipt_13_草地二:13 ↔ 110033226_ipt_02_草地一:2
- 貼合:374 [Mate]: 110033226_ipt_02_草地一:5 ↔ 110033226_ipt_13_草地二:28
- 貼合:375 [Mate]: 110033226_ipt_02_草地一:5 ↔ 110033226_ipt_13_草地二:28
- 貼合:376 [Mate]: 110033226_ipt_02_草地一:5 ↔ 110033226_ipt_13_草地二:28
- 貼合:377 [Mate]: 110033226_ipt_14_草地三:18 ↔ 110033226_ipt_13_草地二:36
- 貼合:378 [Mate]: 110033226_ipt_14_草地三:18 ↔ 110033226_ipt_13_草地二:36
- 貼合:379 [Mate]: 110033226_ipt_14_草地三:18 ↔ 110033226_ipt_13_草地二:36
- 貼合:380 [Mate]: 110033226_ipt_14_草地三:19 ↔ 110033226_ipt_13_草地二:36
- 貼合:381 [Mate]: 110033226_ipt_14_草地三:19 ↔ 110033226_ipt_13_草地二:36
- 貼合:382 [Mate]: 110033226_ipt_14_草地三:19 ↔ 110033226_ipt_13_草地二:36
- 貼合:383 [Mate]: 110033226_ipt_13_草地二:22 ↔ 110033226_ipt_14_草地三:42
- 貼合:384 [Mate]: 110033226_ipt_13_草地二:22 ↔ 110033226_ipt_14_草地三:42
- 貼合:385 [Mate]: 110033226_ipt_13_草地二:22 ↔ 110033226_ipt_14_草地三:42
- 貼合:386 [Mate]: 110033226_ipt_13_草地二:22 ↔ 110033226_ipt_14_草地三:43
- 貼合:387 [Mate]: 110033226_ipt_13_草地二:22 ↔ 110033226_ipt_14_草地三:43
- 貼合:388 [Mate]: 110033226_ipt_14_草地三:42 ↔ 110033226_ipt_14_草地三:43
- 貼合:389 [Mate]: 110033226_ipt_14_草地三:44 ↔ 110033226_ipt_13_草地二:6
- 貼合:390 [Mate]: 110033226_ipt_14_草地三:16 ↔ 110033226_ipt_14_草地三:44
- 貼合:391 [Mate]: 110033226_ipt_14_草地三:44 ↔ 110033226_ipt_13_草地二:6
- 貼合:392 [Mate]: 110033226_ipt_13_草地二:21 ↔ 110033226_ipt_14_草地三:47
- 貼合:393 [Mate]: 110033226_ipt_13_草地二:21 ↔ 110033226_ipt_14_草地三:47
- 貼合:394 [Mate]: 110033226_ipt_14_草地三:46 ↔ 110033226_ipt_13_草地二:5
- 貼合:395 [Mate]: 110033226_ipt_14_草地三:46 ↔ 110033226_ipt_13_草地二:5
- 貼合:396 [Mate]: 110033226_ipt_13_草地二:20 ↔ 110033226_ipt_14_草地三:46
- 貼合:397 [Mate]: 110033226_ipt_14_草地三:45 ↔ 110033226_ipt_13_草地二:6
- 貼合:398 [Mate]: 110033226_ipt_14_草地三:45 ↔ 110033226_ipt_14_草地三:46
- 貼合:399 [Mate]: 110033226_ipt_14_草地三:45 ↔ 110033226_ipt_13_草地二:5
- 貼合:400 [Mate]: 110033226_ipt_15_房子屋頂:1 ↔ 110033226_ipt_07_磚塊樺木(2x1):263
- 貼合:401 [Mate]: 110033226_ipt_15_房子屋頂:1 ↔ 110033226_ipt_07_磚塊樺木(2x1):263
- 貼合:402 [Mate]: 110033226_ipt_15_房子屋頂:1 ↔ 110033226_ipt_06_磚塊樺木(1x1):242
- 貼合:403 [Mate]: 110033226_ipt_07_磚塊樺木(2x1):181 ↔ 110033226_ipt_10_木板條:9
- 貼合:404 [Mate]: 110033226_ipt_07_磚塊樺木(2x1):181 ↔ 110033226_ipt_10_木板條:9
- 貼合:405 [Mate]: 110033226_ipt_07_磚塊樺木(2x1):181 ↔ 110033226_ipt_10_木板條:9
- 貼合:406 [Mate]: 110033226_ipt_24_直條(3x1):2 ↔ 110033226_ipt_10_木板條:11
- 貼合:407 [Mate]: 110033226_ipt_24_直條(3x1):3 ↔ 110033226_ipt_10_木板條:17
- 貼合:409 [Mate]: 110033226_ipt_24_直條(3x1):2 ↔ 110033226_ipt_10_木板條:8
- 貼合:410 [Mate]: 110033226_ipt_24_直條(3x1):2 ↔ 110033226_ipt_10_木板條:8
- 貼合:411 [Mate]: 110033226_ipt_08_平滑面(3x1):37 ↔ 110033226_ipt_10_木板條:15
- 貼合:412 [Mate]: 110033226_ipt_08_平滑面(3x1):37 ↔ 110033226_ipt_10_木板條:15
- 貼合:413 [Mate]: 110033226_ipt_08_平滑面(3x1):37 ↔ 110033226_ipt_10_木板條:12
- 貼合:414 [Mate]: 110033226_ipt_24_直條(3x1):3 ↔ 110033226_ipt_10_木板條:17
- 貼合:416 [Mate]: 110033226_ipt_24_直條(3x1):4 ↔ 110033226_ipt_10_木板條:18
- 貼合:417 [Mate]: 110033226_ipt_24_直條(3x1):5 ↔ 110033226_ipt_10_木板條:12
- 貼合:418 [Mate]: 110033226_ipt_24_直條(3x1):2 ↔ 110033226_ipt_10_木板條:11
- 貼合:419 [Mate]: 110033226_ipt_10_木板條:31 ↔ 110033226_ipt_10_木板條:29
- 貼合:420 [Mate]: 110033226_ipt_10_木板條:31 ↔ 110033226_ipt_10_木板條:29
- 貼合:421 [Mate]: 110033226_ipt_10_木板條:35 ↔ 110033226_ipt_11_樓梯支架:11
- 貼合:422 [Mate]: 110033226_ipt_10_木板條:35 ↔ 110033226_ipt_11_樓梯支架:6
- 貼合:423 [Mate]: 110033226_ipt_10_木板條:35 ↔ 110033226_ipt_11_樓梯支架:6
